# Autodesk Inventor assembly: Rb oven housing
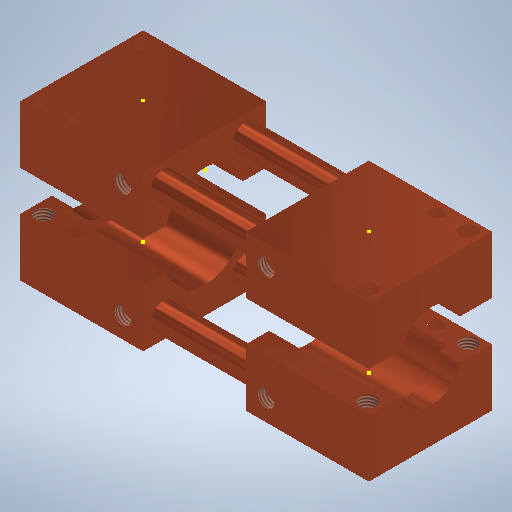
[picture p0: Inventor's stored thumbnail of the model, 512x512]
Saved by Autodesk Inventor 2025.3 (Build 293356000, 356)
## iProperties
Created: 2025-04-24
Part Number: Rb oven housing
Document SubType Name: Assembly
Designer: Verðandi
Author: E. Moreno
Title: Carcasa Horno - Ensamblado
## Documents named in this file (6)
- E:\Users\USER\Documents\GitHub\LAFriOC\Rb oven housing\Rb oven housing.iam
- E:\Users\USER\Documents\GitHub\LAFriOC\Rb oven housing\Rb oven housing bottom-back_front.ipt
- E:\Users\USER\Documents\GitHub\LAFriOC\Rb oven housing\Rb oven housing post.ipt
- E:\Users\USER\Documents\GitHub\LAFriOC\Rb oven housing\Rb oven housing top-back_front.ipt
- E:\Users\USER\Documents\GitHub\LAFriOC\Rb oven housing\Rb oven housing bottom-back_front_MIR_MIR.ipt
- E:\Users\USER\Documents\GitHub\LAFriOC\Rb oven housing\Rb oven housing top-back_front_MIR_MIR.ipt
## Components (8 placed, 5 different names)
1. Rb oven housing bottom-back_front:1 — Flush:1, Flush:2, Flush:3, Mate:3, Mate:4
2. Rb oven housing top-back_front:1 — Flush:1, Flush:2, Flush:3, Mate:1, Mate:2
3. Rb oven housing post:1 — Mate:3, Mate:6
4. Rb oven housing post:2 — Mate:4
5. Rb oven housing post:3 — Mate:2, Mate:5
6. Rb oven housing post:4 — Mate:1
7. Rb oven housing bottom-back_front_MIR_MIR:1 — Mate:6
8. Rb oven housing top-back_front_MIR_MIR:1 — Mate:5
## Relationships (9: Mate 6, Flush 3)
- Flush:1: Rb oven housing bottom-back_front:1 ↔ Rb oven housing top-back_front:1
- Flush:2: Rb oven housing bottom-back_front:1 ↔ Rb oven housing top-back_front:1
- Flush:3: Rb oven housing bottom-back_front:1 ↔ Rb oven housing top-back_front:1
- Mate:1: Rb oven housing top-back_front:1 ↔ Rb oven housing post:4
- Mate:2: Rb oven housing top-back_front:1 ↔ Rb oven housing post:3
- Mate:3: Rb oven housing bottom-back_front:1 ↔ Rb oven housing post:1
- Mate:4: Rb oven housing bottom-back_front:1 ↔ Rb oven housing post:2
- Mate:5 (15 mm): Rb oven housing post:3 ↔ Rb oven housing top-back_front_MIR_MIR:1
- Mate:6 (15 mm): Rb oven housing post:1 ↔ Rb oven housing bottom-back_front_MIR_MIR:1
